# Autodesk Inventor assembly: V-Belt transmission
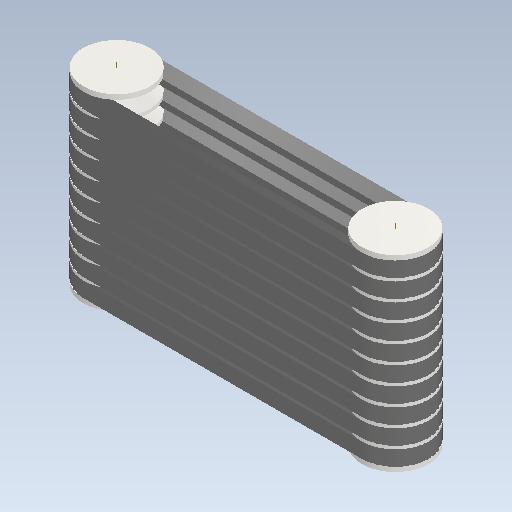
[picture p0: Inventor's stored thumbnail of the model, 512x512]
Saved by Autodesk Inventor 2021.1 (Build 251245000, 245)
## iProperties
ClientObjectVersion: 1
Created: 2021-01-01
Part Number: V-Belt transmission
Document SubType Name: Assembly
Designer: Bolisteward
Author: Bolisteward
## Documents named in this file (4)
- D:\Inventor works\Embebidos\ensamble\Design Accelerator\V-Belt transmission1.iam
- D:\Inventor works\Embebidos\ensamble\Design Accelerator\V-Belt1.ipt
- D:\Inventor works\Embebidos\ensamble\Design Accelerator\Grooved Pulley11.ipt
- D:\Inventor works\Embebidos\ensamble\Design Accelerator\Grooved Pulley21.ipt
## Components (12 placed, 3 different names)
1. Grooved Pulley1:1 — Flush:1, Mate:1, Rotation:1
2. Grooved Pulley2:1 — Flush:2, Mate:2, Rotation:1
3. V-Belt:1 — Flush:1, Mate:1, Flush:2, Mate:2
4. V-Belt:2
5. V-Belt:3
6. V-Belt:4
7. V-Belt:5
8. V-Belt:6
9. V-Belt:7
10. V-Belt:8
11. V-Belt:9
12. V-Belt:10
## Component patterns: (10 elements, first: V-Belt:1)
## Relationships (5: Flush 2, Mate 2, RelateRotation 1)
- Flush:1: Grooved Pulley1:1 ↔ V-Belt:1
- Mate:1: Grooved Pulley1:1 ↔ V-Belt:1
- Flush:2: Grooved Pulley2:1 ↔ V-Belt:1
- Mate:2: Grooved Pulley2:1 ↔ V-Belt:1
- Rotation:1 [RelateRotation] (1 ul): Grooved Pulley1:1 ↔ Grooved Pulley2:1
